# Autodesk Inventor assembly: AX-12A
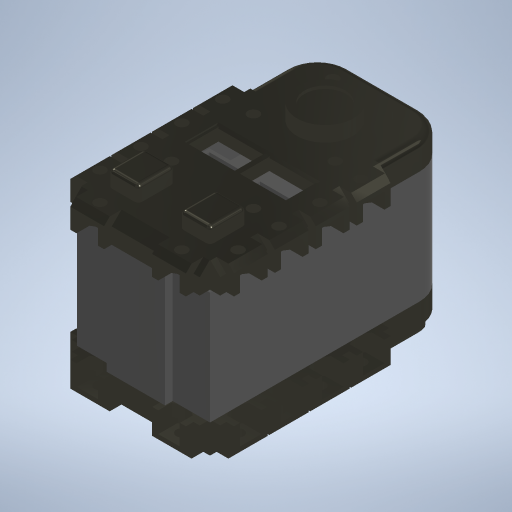
[picture p0: Inventor's stored thumbnail of the model, 512x512]
Saved by Autodesk Inventor 2024.2 (Build 282272000, 272)
## iProperties
Created: 2025-09-29
Part Number: AX-12A
Document SubType Name: Assembly
Designer: Admin
Author: Admin
## Documents named in this file (4)
- C:\Users\Admin\Documents\GitHub\ManipuladorCartesiano\DiseñoMecánico\Assemblies\AX-12A.iam
- C:\Users\Admin\Documents\GitHub\ManipuladorCartesiano\DiseñoMecánico\Motors\DynamixelAX12A\Pieces\AX12 Back.STEP.ipt
- C:\Users\Admin\Documents\GitHub\ManipuladorCartesiano\DiseñoMecánico\Motors\DynamixelAX12A\Pieces\AX12 middle.STEP.ipt
- C:\Users\Admin\Documents\GitHub\ManipuladorCartesiano\DiseñoMecánico\Motors\DynamixelAX12A\Pieces\AX12 Front.STEP.ipt
## Components (3 placed, 3 different names)
1. AX12 Back.STEP:1 — Mate:1, Flush:1, Flush:2
2. AX12 middle.STEP:1 — Mate:1, Flush:1, Flush:2, Mate:2, Flush:3, Flush:4
3. AX12 Front.STEP:1 — Mate:2, Flush:3, Flush:4
## Relationships (6: Flush 4, Mate 2)
- Mate:1: AX12 Back.STEP:1 ↔ AX12 middle.STEP:1
- Flush:1: AX12 Back.STEP:1 ↔ AX12 middle.STEP:1
- Flush:2: AX12 Back.STEP:1 ↔ AX12 middle.STEP:1
- Mate:2: AX12 middle.STEP:1 ↔ AX12 Front.STEP:1
- Flush:3: AX12 middle.STEP:1 ↔ AX12 Front.STEP:1
- Flush:4: AX12 middle.STEP:1 ↔ AX12 Front.STEP:1
